# Autodesk Inventor assembly: 6 bar
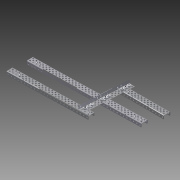
[picture p0: Inventor's stored thumbnail of the model, 180x180]
Saved by Autodesk Inventor 2014 (Build 180170000, 170)
## iProperties
Created: 2013-09-14
Part Number: 6 bar
Document SubType Name: Assembly
Designer: Ryan
Author: Ryan
## Documents named in this file (9)
- C:\Users\Ryan\Desktop\sw\6 bar\6 bar.iam
- C:\Users\Ryan\Desktop\sw\lib\Aperture VEX CAD Library\Metal\C Channel\2 x 35.ipt
- C:\Users\Ryan\Desktop\sw\lib\Aperture VEX CAD Library\Metal\C Channel\2 x 25.ipt
- C:\Users\Ryan\Desktop\sw\lib\Aperture VEX CAD Library\Metal\C Channel\2 x 15.ipt
- C:\Users\Ryan\Desktop\sw\lib\Aperture VEX CAD Library\Bearing Blocks\Bearing Block.ipt
- C:\Users\Ryan\Desktop\sw\lib\Aperture VEX CAD Library\Hardware\8-32\8-32_.375.ipt
- C:\Users\Ryan\Desktop\sw\lib\Aperture VEX CAD Library\Spacers\SPACER-0500-0125.ipt
- C:\Users\Ryan\Desktop\sw\lib\Aperture VEX CAD Library\Hardware\8-32\8-32_.875.ipt
- C:\Users\Ryan\Desktop\sw\lib\Aperture VEX CAD Library\Hardware\8-32\8-32 Nylock.ipt
## Components (38 placed, 8 different names)
1. 2 x 35:1 — Mate:39, Mate:40, Mate:41, Mate:42, Mate:45, Mate:79, Mate:80, Mate:81, Mate:82, Mate:87, Mate:89, Mate:100, Mate:103, Mate:104, Mate:105, Mate:106, Mate:107, Mate:108
2. 2 x 25:1 — Mate:50, Mate:51, Mate:52, Mate:53, Mate:60, Mate:91, Mate:92, Mate:93, Mate:94, Mate:98, Mate:99
3. 2 x 15:1 — Mate:1, Mate:10, Mate:12, Mate:14, Mate:15, Mate:16, Mate:17, Mate:83
4. Bearing Block:1 — Mate:1, Mate:9, Mate:11, Mate:13, Mate:26, Mate:64
5. 2 x 15:2 — Mate:20, Mate:21, Mate:22, Mate:23, Mate:24, Mate:25, Mate:27, Mate:30, Mate:32, Mate:34, Mate:44, Mate:54, Mate:56, Mate:57, Mate:59, Mate:62, Mate:84, Mate:85, Mate:86
6. SPACER-0500-0125:1 — Mate:9, Mate:10, Mate:27
7. 8-32_.375:3 — Mate:11, Mate:12, Mate:15, Mate:16
8. 8-32_.375:4 — Mate:13, Mate:14, Mate:17, Mate:83
9. Bearing Block:4 — Mate:30, Mate:55, Mate:58
10. 8-32_.375:9 — Mate:32, Mate:34, Mate:56
11. Bearing Block:5 — Mate:38, Mate:39, Mate:43, Mate:46, Mate:65, Mate:67
12. 8-32_.375:11 — Flush:1, Mate:42, Mate:108
13. 8-32_.375:12 — Mate:38, Flush:1, Mate:40, Mate:41, Mate:88
14. SPACER-0500-0125:2 — Mate:44, Mate:45, Mate:46
15. Bearing Block:6 — Mate:50, Mate:58, Mate:61, Mate:66, Mate:68
16. 8-32_.375:13 — Mate:51, Mate:52
17. 8-32_.375:14 — Mate:53
18. 8-32_.375:15 — Mate:54, Mate:55, Mate:57, Mate:62
19. SPACER-0500-0125:3 — Mate:59, Mate:60, Mate:61
20. 8-32_.875:1 — Mate:63, Mate:64
21. 8-32_.875:2 — Mate:66, Mate:68
22. 8-32_.875:3 — Mate:65, Mate:67
23. Bearing Block:8 — Mate:82
24. 8-32_.375:18 — Mate:79, Mate:80
25. 8-32_.375:19 — Mate:81, Mate:87
26. 8-32 Nylock:1 — Mate:88, Mate:89
27. Bearing Block:9 — Mate:91, Mate:92, Mate:93, Mate:94, Mate:95, Mate:97
28. 8-32_.375:20 — Mate:95, Mate:99
29. 8-32_.375:21 — Mate:97, Mate:98
30. Bearing Block:10 — Mate:100, Mate:101, Mate:102
31. 8-32_.375:22 — Mate:101, Mate:103, Mate:105, Mate:106
32. 8-32_.375:23 — Mate:102, Mate:104, Mate:107
33. 8-32_.375:6 — Mate:22, Mate:25, Mate:84, Mate:85, Mate:86
34. Bearing Block:2 — Mate:20, Mate:26, Mate:63
35. 8-32_.375:5 — Mate:21, Mate:23, Mate:24
36. 8-32_.375:7
37. Bearing Block:3 — Mate:43
38. 8-32_.375:8
## Component patterns: (2 elements, first: 8-32_.375:6 + Bearing Block:2 + 8-32_.375:5)
## Relationships (91: Mate 88, Flush 3)
- Mate:1: 2 x 15:1 ↔ Bearing Block:1
- Mate:9: Bearing Block:1 ↔ SPACER-0500-0125:1
- Mate:10: 2 x 15:1 ↔ SPACER-0500-0125:1
- Mate:11: Bearing Block:1 ↔ 8-32_.375:3
- Mate:12: 2 x 15:1 ↔ 8-32_.375:3
- Mate:13: Bearing Block:1 ↔ 8-32_.375:4
- Mate:14: 2 x 15:1 ↔ 8-32_.375:4
- Mate:15 (2.3114 mm): 2 x 15:1 ↔ 8-32_.375:3
- Mate:16 (2.3114 mm): 2 x 15:1 ↔ 8-32_.375:3
- Mate:17 (2.3114 mm): 2 x 15:1 ↔ 8-32_.375:4
- [Mate]: Bearing Block:2 ↔ 8-32_.375:5
- [Mate]: 8-32_.375:6 ↔ Bearing Block:2
- Mate:20: 2 x 15:2 ↔ Bearing Block:2
- Mate:21: 2 x 15:2 ↔ 8-32_.375:5
- Mate:22: 2 x 15:2 ↔ 8-32_.375:6
- Mate:23 (2.3114 mm): 2 x 15:2 ↔ 8-32_.375:5
- Mate:24 (2.3114 mm): 2 x 15:2 ↔ 8-32_.375:5
- Mate:25 (2.3114 mm): 2 x 15:2 ↔ 8-32_.375:6
- Mate:26: Bearing Block:1 ↔ Bearing Block:2
- Mate:27: 2 x 15:2 ↔ SPACER-0500-0125:1
- [Mate]: Bearing Block:4 ↔ 8-32_.375:9
- Mate:30: 2 x 15:2 ↔ Bearing Block:4
- Mate:32: 2 x 15:2 ↔ 8-32_.375:9
- Mate:34 (2.3114 mm): 2 x 15:2 ↔ 8-32_.375:9
- [Mate]: Bearing Block:5 ↔ 8-32_.375:11
- [Mate]: Bearing Block:5 ↔ 8-32_.375:12
- Mate:38 (1.1684 mm): Bearing Block:5 ↔ 8-32_.375:12
- Flush:1: 8-32_.375:11 ↔ 8-32_.375:12
- Mate:39: 2 x 35:1 ↔ Bearing Block:5
- Mate:40 (2.3114 mm): 2 x 35:1 ↔ 8-32_.375:12
- Mate:41 (2.3114 mm): 2 x 35:1 ↔ 8-32_.375:12
- Mate:42 (2.3114 mm): 2 x 35:1 ↔ 8-32_.375:11
- Mate:43: Bearing Block:5 ↔ Bearing Block:3
- Mate:44: 2 x 15:2 ↔ SPACER-0500-0125:2
- Mate:45: 2 x 35:1 ↔ SPACER-0500-0125:2
- Mate:46: Bearing Block:5 ↔ SPACER-0500-0125:2
- [Mate]: Bearing Block:6 ↔ 8-32_.375:13
- [Mate]: Bearing Block:6 ↔ 8-32_.375:14
- [Mate] (1.1684 mm): Bearing Block:6 ↔ 8-32_.375:14
- [Flush]: 8-32_.375:13 ↔ 8-32_.375:14
- Mate:50: 2 x 25:1 ↔ Bearing Block:6
- Mate:51 (2.3114 mm): 2 x 25:1 ↔ 8-32_.375:13
- Mate:52 (2.3114 mm): 2 x 25:1 ↔ 8-32_.375:13
- Mate:53 (2.3114 mm): 2 x 25:1 ↔ 8-32_.375:14
- Mate:54: 2 x 15:2 ↔ 8-32_.375:15
- Mate:55: Bearing Block:4 ↔ 8-32_.375:15
- Mate:56 (2.3114 mm): 2 x 15:2 ↔ 8-32_.375:9
- Mate:57 (2.3114 mm): 2 x 15:2 ↔ 8-32_.375:15
- Mate:58: Bearing Block:4 ↔ Bearing Block:6
- Mate:59: 2 x 15:2 ↔ SPACER-0500-0125:3
- Mate:60: 2 x 25:1 ↔ SPACER-0500-0125:3
- Mate:61: Bearing Block:6 ↔ SPACER-0500-0125:3
- Mate:62 (2.3114 mm): 2 x 15:2 ↔ 8-32_.375:15
- Mate:63: 8-32_.875:1 ↔ Bearing Block:2
- Mate:64: Bearing Block:1 ↔ 8-32_.875:1
- Mate:65: Bearing Block:5 ↔ 8-32_.875:3
- Mate:66: Bearing Block:6 ↔ 8-32_.875:2
- Mate:67: Bearing Block:5 ↔ 8-32_.875:3
- Mate:68: Bearing Block:6 ↔ 8-32_.875:2
- [Mate]: Bearing Block:8 ↔ 8-32_.375:18
- [Mate]: Bearing Block:8 ↔ 8-32_.375:19
- [Mate] (1.1684 mm): Bearing Block:8 ↔ 8-32_.375:19
- [Flush]: 8-32_.375:18 ↔ 8-32_.375:19
- Mate:79 (2.3114 mm): 2 x 35:1 ↔ 8-32_.375:18
- Mate:80 (2.3114 mm): 2 x 35:1 ↔ 8-32_.375:18
- Mate:81 (2.3114 mm): 2 x 35:1 ↔ 8-32_.375:19
- Mate:82: 2 x 35:1 ↔ Bearing Block:8
- Mate:83 (2.3114 mm): 2 x 15:1 ↔ 8-32_.375:4
- Mate:84 (2.3114 mm): 2 x 15:2 ↔ 8-32_.375:6
- Mate:85 (2.3114 mm): 2 x 15:2 ↔ 8-32_.375:6
- Mate:86 (2.3114 mm): 2 x 15:2 ↔ 8-32_.375:6
- Mate:87 (2.3114 mm): 2 x 35:1 ↔ 8-32_.375:19
- Mate:88: 8-32_.375:12 ↔ 8-32 Nylock:1
- Mate:89: 2 x 35:1 ↔ 8-32 Nylock:1
- Mate:91: 2 x 25:1 ↔ Bearing Block:9
- Mate:92 (2.3114 mm): 2 x 25:1 ↔ Bearing Block:9
- Mate:93 (2.3114 mm): 2 x 25:1 ↔ Bearing Block:9
- Mate:94 (2.3114 mm): 2 x 25:1 ↔ Bearing Block:9
- Mate:95: Bearing Block:9 ↔ 8-32_.375:20
- Mate:97: Bearing Block:9 ↔ 8-32_.375:21
- Mate:98: 2 x 25:1 ↔ 8-32_.375:21
- Mate:99: 2 x 25:1 ↔ 8-32_.375:20
- Mate:100: 2 x 35:1 ↔ Bearing Block:10
- Mate:101: Bearing Block:10 ↔ 8-32_.375:22
- Mate:102: Bearing Block:10 ↔ 8-32_.375:23
- Mate:103: 2 x 35:1 ↔ 8-32_.375:22
- Mate:104: 2 x 35:1 ↔ 8-32_.375:23
- Mate:105 (2.3114 mm): 2 x 35:1 ↔ 8-32_.375:22
- Mate:106 (2.3114 mm): 2 x 35:1 ↔ 8-32_.375:22
- Mate:107 (2.3114 mm): 2 x 35:1 ↔ 8-32_.375:23
- Mate:108 (2.3114 mm): 2 x 35:1 ↔ 8-32_.375:11
## Named parameters: q = 2.3114 mm, d21_d14 = 0 mm, d22_d16 = 0 mm, d40_d21_d14 = 0 mm, d48_d21_d14 = 0 mm, d49_d22_d16 = 0 mm, d60_d50 = 1.1684 mm, d61_d51 = 0 mm, d62_d48_d21_d14 = 0 mm, d63_d49_d22_d16 = 0 mm, d111_d103_d60_d50 = 1.1684 mm, d112_d104_d61_d51 = 0 mm, d113_d105_d62_d48_d21_d14 = 0 mm, d114_d106_d63_d49_d22_d16 = 0 mm
